# Autodesk Inventor assembly: ASY SLM 179 top funnel 1200 50-90_1000x90
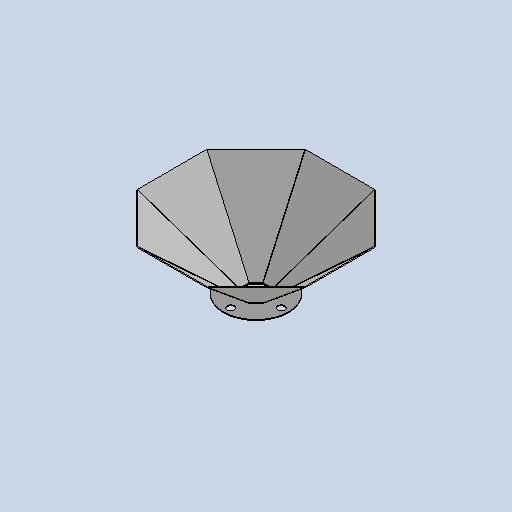
[picture p0: Inventor's stored thumbnail of the model, 512x512]
Saved by Autodesk Inventor 2025.3 (Build 293356030, 356C)
## iProperties
Created: 2025-07-11
Part Number: ASY SLM 179 top funnel 1200 50-90_1000x90
Document SubType Name: Assembly
Designer: user
Mass: 3988.24 g
Surface Area: 4860.23 cm^2
Volume: 498.53 cm^3
Density: 8 g/cm^3
Author: user
## Documents named in this file (3)
- C:\Users\admin\Documents\Inventor\NDA-Nyyda\ASY PNS 179 top funnel 1200 50-90_1000x90.iam
- C:\Users\admin\Documents\Inventor\NDA-Nyyda\PNS 1792  funnel FLANGE 1200 50-90_1000x90.ipt
- C:\Users\admin\Documents\Inventor\NDA-Nyyda\PNS 1791 top funnel 1200 50-90_1000x90.ipt
## Components (3 placed, 2 different names)
1. PNS 1792  funnel FLANGE 1200 50-90_1000x90:1 — Mate:2, Mate:1, Mate:4, Mate:3
2. PNS 1791 top funnel 1200 50-90_1000x90:1 — Mate:2, Mate:1, Mate:5
3. PNS 1791 top funnel 1200 50-90_1000x90:2 — Mate:5, Mate:4, Mate:3
## Relationships (5: Mate 5)
- Mate:2: PNS 1792  funnel FLANGE 1200 50-90_1000x90:1 ↔ PNS 1791 top funnel 1200 50-90_1000x90:1
- Mate:1: PNS 1792  funnel FLANGE 1200 50-90_1000x90:1 ↔ PNS 1791 top funnel 1200 50-90_1000x90:1
- Mate:5: PNS 1791 top funnel 1200 50-90_1000x90:1 ↔ PNS 1791 top funnel 1200 50-90_1000x90:2
- Mate:4: PNS 1792  funnel FLANGE 1200 50-90_1000x90:1 ↔ PNS 1791 top funnel 1200 50-90_1000x90:2
- Mate:3: PNS 1792  funnel FLANGE 1200 50-90_1000x90:1 ↔ PNS 1791 top funnel 1200 50-90_1000x90:2
